# Autodesk Inventor assembly: Ensamble
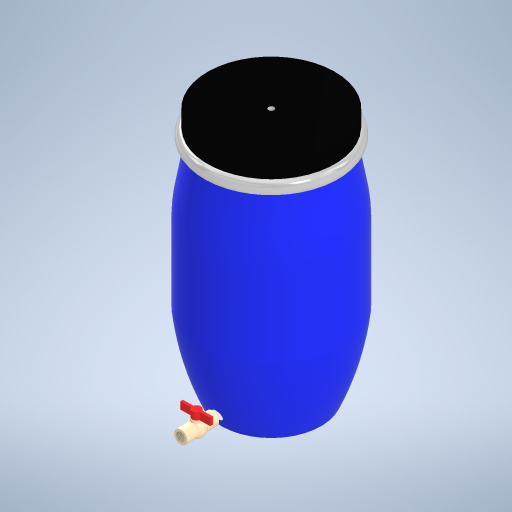
[picture p0: Inventor's stored thumbnail of the model, 512x512]
Saved by Autodesk Inventor 2024 (Build 280153000, 153)
## iProperties
Created: 2024-04-30
Part Number: Ensamble
Document SubType Name: Assembly
Designer: alexa
Author: alexa
## Documents named in this file (4)
- C:\Users\alexa\OneDrive\Escritorio\Biogas\Ensamble.iam
- C:\Users\alexa\OneDrive\Escritorio\Biogas\Contenedor.ipt
- C:\Users\alexa\OneDrive\Escritorio\Biogas\AcopleHembra.ipt
- C:\Users\alexa\OneDrive\Escritorio\Biogas\LlaveDesecho.ipt
## Components (3 placed, 3 different names)
1. Contenedor:1 — Mate:1, Mate:2, Tangent:1, Mate:5, Mate:6
2. AcopleHembra:1 — Mate:1, Tangent:1
3. LlaveDesecho:1 — Mate:5, Mate:6
## Relationships (5: Mate 4, Tangent 1)
- Mate:1: Contenedor:1 ↔ AcopleHembra:1
- Mate:2: Contenedor:1
- Tangent:1: Contenedor:1 ↔ AcopleHembra:1
- Mate:5: Contenedor:1 ↔ LlaveDesecho:1
- Mate:6: Contenedor:1 ↔ LlaveDesecho:1
